# Autodesk Inventor assembly: Assembly2
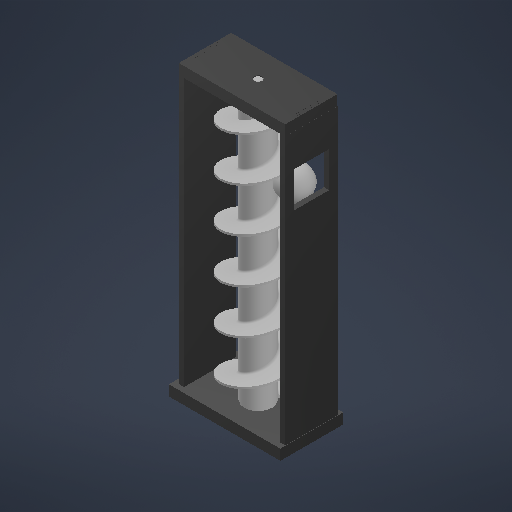
[picture p0: Inventor's stored thumbnail of the model, 512x512]
Saved by Autodesk Inventor 2026.2 (Build 302298000, 298)
## iProperties
Created: 2026-03-02
Part Number: Assembly2
Document SubType Name: Assembly
Designer: shahd
Author: shahd
## Documents named in this file (8)
- C:\Users\danda\BOM-project\Project\CAD\Lifting\Lifting Mechanism\Assembly2.iam
- C:\Users\danda\BOM-project\Project\CAD\Lifting\Lifting Mechanism\Part3.ipt
- C:\Users\danda\BOM-project\Project\CAD\Lifting\Lifting Mechanism\Lifting Mechanism.ipt
- C:\Users\danda\BOM-project\Project\CAD\Lifting\Lifting Mechanism\base.ipt
- C:\Users\danda\BOM-project\Project\CAD\Lifting\Lifting Mechanism\partttt.ipt
- C:\Users\danda\BOM-project\Project\CAD\Lifting\Lifting Mechanism\coupler.ipt
- C:\Users\danda\BOM-project\Project\CAD\Lifting\Lifting Mechanism\ball.ipt
- C:\Users\danda\BOM-project\Project\CAD\Lifting\Lifting Mechanism\Part4.ipt
## Components (7 placed, 7 different names)
1. Part3:1 — Flush:19, Flush:20, Flush:21
2. Lifting Mechanism:1 — Mate:8, Flush:17, Mate:19, Tangent:1, Mate:22, Mate:36, Mate:41
3. base:1 — Mate:8, Mate:19, Mate:22, Mate:28, Mate:29, Mate:31, Mate:32, Mate:37
4. partttt:1 — Mate:28, Mate:29, Mate:42, Flush:18
5. ball:1 — Tangent:1
6. coupler:1 — Mate:36, Mate:37
7. Part4:1 — Mate:41, Mate:42, Flush:18, Flush:19, Flush:20, Flush:21
## Relationships (17: Mate 11, Flush 5, Tangent 1)
- Mate:8: Lifting Mechanism:1 ↔ base:1
- Flush:17 (-300 mm): Lifting Mechanism:1
- Mate:19: Lifting Mechanism:1 ↔ base:1
- Tangent:1: Lifting Mechanism:1 ↔ ball:1
- Mate:22: Lifting Mechanism:1 ↔ base:1
- Mate:28: base:1 ↔ partttt:1
- Mate:29: base:1 ↔ partttt:1
- Mate:31: base:1
- Mate:32: base:1
- Mate:36: Lifting Mechanism:1 ↔ coupler:1
- Mate:37: base:1 ↔ coupler:1
- Mate:41: Lifting Mechanism:1 ↔ Part4:1
- Mate:42: partttt:1 ↔ Part4:1
- Flush:18: partttt:1 ↔ Part4:1
- Flush:19: Part3:1 ↔ Part4:1
- Flush:20: Part3:1 ↔ Part4:1
- Flush:21: Part3:1 ↔ Part4:1
